# Autodesk Inventor assembly: 2x4
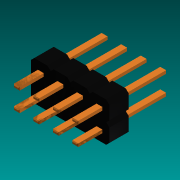
[picture p0: Inventor's stored thumbnail of the model, 180x180]
Saved by Autodesk Inventor 2015 (Build 190159000, 159)
## iProperties
Created: 2014-07-19
Part Number: 2x4
Document SubType Name: Assembly
Designer: Sawaiz Syed
Author: Sawaiz Syed
## Documents named in this file (2)
- C:\Users\Admin\SkyDrive\Classes\College\Semester 6\Research Project\Hardware\Transmitter 3D\Inventor\Radiation Dector\2.54 Breakaway\2x4.iam
- C:\Users\Admin\SkyDrive\Classes\College\Semester 6\Research Project\Hardware\Transmitter 3D\Inventor\Radiation Dector\2.54 Breakaway\1x1.iam
## Components (8 placed, 1 different names)
1. 1x1:1 [sub-assembly]
2. 1x1:2 [sub-assembly]
3. 1x1:3 [sub-assembly]
4. 1x1:4 [sub-assembly]
5. 1x1:5 [sub-assembly]
6. 1x1:6 [sub-assembly]
7. 1x1:7 [sub-assembly]
8. 1x1:8 [sub-assembly]
## Component patterns: (8 elements, first: 1x1:1)
